# Autodesk Inventor assembly: assy-shooter_urdf_all
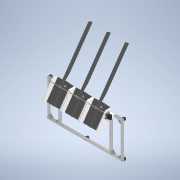
[picture p0: Inventor's stored thumbnail of the model, 180x180]
Saved by Autodesk Inventor 2022 (Build 260153000, 153)
## iProperties
Created: 2021-10-15
Part Number: assy-shooter_urdf_all
Document SubType Name: Assembly
Designer: yuto6
Author: yuto6
## Documents named in this file (4)
- C:\Users\yuto6\Documents\catchrobo_hardware\assy-shooter\assy-shooter_urdf_all.iam
- C:\Users\yuto6\Documents\catchrobo_hardware\assy-shooter\assy-shooter_urdf_base_fixed_axis.iam
- C:\Users\yuto6\Documents\catchrobo_hardware\assy-shooter\assy-shooter_urdf_guide.iam
- C:\Users\yuto6\Documents\catchrobo_hardware\assy-shooter\assy-shooter_urdf_sorter.iam
## Components (5 placed, 3 different names)
1. assy-shooter_urdf_base_fixed_axis:1 [sub-assembly] — メイト:1, メイト:2, メイト:3, メイト:4, メイト:5, メイト:6, メイト:7, メイト:8, guide, sorter1, sorter2, sorter3
2. assy-shooter_urdf_guide:1 [sub-assembly] — メイト:1, メイト:2, guide
3. assy-shooter_urdf_sorter:1 [sub-assembly] — メイト:3, メイト:6, sorter1
4. assy-shooter_urdf_sorter:2 [sub-assembly] — メイト:4, メイト:7, sorter2
5. assy-shooter_urdf_sorter:3 [sub-assembly] — メイト:5, メイト:8, sorter3
## Relationships (12: Mate 8, Angle 4)
- メイト:1 [Mate]: assy-shooter_urdf_base_fixed_axis:1 ↔ assy-shooter_urdf_guide:1
- メイト:2 [Mate]: assy-shooter_urdf_base_fixed_axis:1 ↔ assy-shooter_urdf_guide:1
- メイト:3 [Mate]: assy-shooter_urdf_base_fixed_axis:1 ↔ assy-shooter_urdf_sorter:1
- メイト:4 [Mate]: assy-shooter_urdf_base_fixed_axis:1 ↔ assy-shooter_urdf_sorter:2
- メイト:5 [Mate]: assy-shooter_urdf_base_fixed_axis:1 ↔ assy-shooter_urdf_sorter:3
- メイト:6 [Mate]: assy-shooter_urdf_base_fixed_axis:1 ↔ assy-shooter_urdf_sorter:1
- メイト:7 [Mate]: assy-shooter_urdf_base_fixed_axis:1 ↔ assy-shooter_urdf_sorter:2
- メイト:8 [Mate]: assy-shooter_urdf_base_fixed_axis:1 ↔ assy-shooter_urdf_sorter:3
- guide [Angle] (0 deg): assy-shooter_urdf_base_fixed_axis:1 ↔ assy-shooter_urdf_guide:1
- sorter1 [Angle] (0 deg): assy-shooter_urdf_base_fixed_axis:1 ↔ assy-shooter_urdf_sorter:1
- sorter2 [Angle] (0 deg): assy-shooter_urdf_base_fixed_axis:1 ↔ assy-shooter_urdf_sorter:2
- sorter3 [Angle] (0 deg): assy-shooter_urdf_base_fixed_axis:1 ↔ assy-shooter_urdf_sorter:3
